# Autodesk Inventor assembly: 6_right_Arm_joint
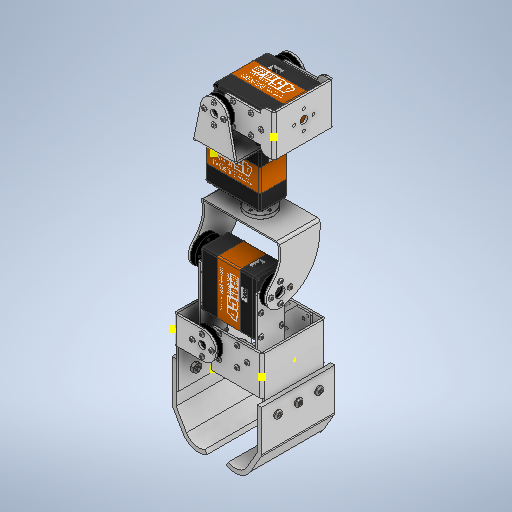
[picture p0: Inventor's stored thumbnail of the model, 512x512]
Saved by Autodesk Inventor 2026.1 (Build 301233020, 233B)
## iProperties
Created: 2026-01-04
Part Number: 6_right_Arm_joint
Document SubType Name: Assembly
Designer: aa992
Author: aa992
## Documents named in this file (18)
- C:\Users\aa992\OneDrive\Desktop\RHp_Humanoid_ver1\Assembly\6_right_Arm_joint.iam
- C:\Users\aa992\OneDrive\Desktop\RHp_Humanoid_ver1\Part\Frame\Arm\axis_18_top_frame.ipt
- C:\Users\aa992\OneDrive\Desktop\RHp_Humanoid_ver1\Part\HTD-45H, Horn\HTD-45H\HTD-45H.iam
- C:\Users\aa992\OneDrive\Desktop\RHp_Humanoid_ver1\Part\HTD-45H, Horn\Horn\Bottom Horn.ipt
- C:\Users\aa992\OneDrive\Desktop\RHp_Humanoid_ver1\Part\HTD-45H, Horn\Horn\Top Horn.ipt
- C:\Users\aa992\OneDrive\Desktop\RHp_Humanoid_ver1\Part\Frame\Arm\axis_19_bottom_frame.ipt
- C:\Users\aa992\OneDrive\Desktop\RHp_Humanoid_ver1\Part\HTD-45H, Horn\Horn\Top Horn silver.ipt
- C:\Users\aa992\OneDrive\Desktop\RHp_Humanoid_ver1\Part\Frame\Arm\axis_20_bottom_frame.ipt
- C:\Users\aa992\OneDrive\Desktop\RHp_Humanoid_ver1\Part\Frame\Arm\axis_21_top_frame.ipt
- C:\Users\aa992\OneDrive\Desktop\RHp_Humanoid_ver1\Part\Frame\Arm\axis_21_bottom_frame.ipt
- C:\Users\aa992\OneDrive\Desktop\RHp_Humanoid_ver1\Part\Frame\Arm\axis_22_top_frame.ipt
- C:\Users\aa992\OneDrive\Desktop\RHp_Humanoid_ver1\Part\Frame\Arm\axis_22_bottom_frame.ipt
- C:\Users\aa992\OneDrive\Desktop\RHp_Humanoid_ver1\Part\Frame\Arm\gripper_frame.ipt
- C:\Users\aa992\OneDrive\Desktop\RHp_Humanoid_ver1\Part\Bolt, Bearing, Nut, Washer\볼트, 너트\M2x4 Bolt.ipt
- C:\Users\aa992\OneDrive\Desktop\RHp_Humanoid_ver1\Part\Bolt, Bearing, Nut, Washer\볼트, 너트\M2x6 Bolt.ipt
- C:\Users\aa992\OneDrive\Desktop\RHp_Humanoid_ver1\Part\Bolt, Bearing, Nut, Washer\볼트, 너트\M3x6 Bolt.ipt
- C:\Users\aa992\OneDrive\Desktop\RHp_Humanoid_ver1\Part\Bolt, Bearing, Nut, Washer\볼트, 너트\M3 Nut.ipt
- C:\Users\aa992\OneDrive\Desktop\RHp_Humanoid_ver1\Part\Bolt, Bearing, Nut, Washer\볼트, 너트\M3x8 Bolt.ipt
## Components (99 placed, 17 different names)
1. axis_18_top_frame:1 — Flush:2, Mate:2, Flush:3, Rigid:1, Rigid:21, Rigid:22, Rigid:23, Rigid:24, Rigid:25, Rigid:26, Rigid:27, Rigid:28, Rigid:29
2. HTD-45H:1 [sub-assembly] — Rigid:1, Rotational:1, Rigid:2
3. Bottom Horn:1 — Rigid:2
4. Top Horn:1 — Rotational:1, Rigid:16
5. axis_19_bottom_frame:1 — Rigid:4, Rigid:16, Rigid:17, Rigid:18, Rigid:19, Rigid:20, Rigid:30, Rigid:31, Rigid:32, Rigid:33, Rigid:34, Rigid:35, Rigid:36, Rigid:37
6. HTD-45H:2 [sub-assembly] — Rigid:4, Rotational:2
7. Top Horn silver:1 — Rotational:2, Rigid:5
8. axis_20_bottom_frame:1 — Rigid:5, Rigid:6, Rigid:7, Rigid:38, Rigid:39, Rigid:40, Rigid:41, Rigid:42, Rigid:43, Rigid:44, Rigid:45, Rigid:46, Rigid:47, Rigid:48, Rigid:49
9. Top Horn:2 — Rigid:6, Rotational:3
10. Bottom Horn:2 — Rigid:7
11. HTD-45H:3 [sub-assembly] — Rotational:3, Rigid:8
12. axis_21_top_frame:1 — Rigid:8, Rigid:9, Rigid:50, Rigid:51, Rigid:52, Rigid:53, Rigid:54, Rigid:55, Rigid:56, Rigid:57, Rigid:58, Rigid:76, Rigid:77, Rigid:78, Rigid:79
13. axis_21_bottom_frame:1 — Rigid:9, Rigid:10, Rigid:12, Rigid:80, Rigid:81, Rigid:82, Rigid:83
14. HTD-45H:4 [sub-assembly] — Rigid:10, Rotational:4, Rigid:11
15. Top Horn:3 — Rotational:4, Rigid:13
16. Bottom Horn:3 — Rigid:11
17. axis_22_top_frame:1 — Rigid:12, Rigid:15, Rigid:63, Rigid:64, Rigid:65, Rigid:66, Rigid:67, Rigid:72, Rigid:73, Rigid:74, Rigid:75, Rigid:93, Rigid:94, Rigid:95
18. axis_22_bottom_frame:1 — Rigid:13, Rigid:14, Rigid:59, Rigid:60, Rigid:61, Rigid:62, Rigid:68, Rigid:69, Rigid:70, Rigid:71, Rigid:90, Rigid:91, Rigid:92
19. gripper_frame:1 — Rigid:14, Rigid:84, Rigid:85, Rigid:86
20. gripper_frame:2 — Rigid:15, Rigid:87, Rigid:88, Rigid:89
21. M2x4 Bolt:1 — Rigid:18
22. M2x4 Bolt:2 — Rigid:17
23. M2x4 Bolt:3 — Rigid:25
24. M2x4 Bolt:4 — Rigid:22
25. M2x4 Bolt:5 — Rigid:20
26. M2x4 Bolt:6 — Rigid:19
27. M2x4 Bolt:7 — Rigid:23
28. M2x4 Bolt:8 — Rigid:21
29. M2x4 Bolt:9 — Rigid:24
30. M2x4 Bolt:10 — Rigid:29
31. M2x4 Bolt:11 — Rigid:26
32. M2x4 Bolt:12 — Rigid:31
33. M2x4 Bolt:13 — Rigid:27
34. M2x4 Bolt:14 — Rigid:32
35. M2x4 Bolt:15 — Rigid:28
36. M2x4 Bolt:16 — Rigid:33
37. M2x4 Bolt:17 — Rigid:30
38. M2x4 Bolt:18 — Rigid:35
39. M2x4 Bolt:19 — Rigid:34
40. M2x4 Bolt:20 — Rigid:37
41. M2x4 Bolt:21 — Rigid:36
42. M2x4 Bolt:22 — Rigid:41
43. M2x4 Bolt:23 — Rigid:44
44. M2x4 Bolt:24 — Rigid:42
45. M2x4 Bolt:25 — Rigid:45
46. M2x4 Bolt:26 — Rigid:40
47. M2x4 Bolt:27 — Rigid:43
48. M2x4 Bolt:28 — Rigid:38
49. M2x4 Bolt:29 — Rigid:39
50. M2x4 Bolt:30 — Rigid:48
51. M2x4 Bolt:31 — Rigid:46
52. M2x4 Bolt:32 — Rigid:49
53. M2x4 Bolt:33 — Rigid:50
54. M2x4 Bolt:34 — Rigid:52
55. M2x4 Bolt:35 — Rigid:47
56. M2x4 Bolt:36 — Rigid:53
57. M2x4 Bolt:37 — Rigid:51
58. M2x4 Bolt:38 — Rigid:54
59. M2x4 Bolt:39 — Rigid:57
60. M2x4 Bolt:40 — Rigid:55
61. M2x4 Bolt:41 — Rigid:58
62. M2x4 Bolt:42 — Rigid:56
63. M2x4 Bolt:43 — Rigid:60
64. M2x4 Bolt:44 — Rigid:59
65. M2x4 Bolt:45 — Rigid:62
66. M2x4 Bolt:46 — Rigid:61
67. M2x6 Bolt:1 — Rigid:64
68. M2x6 Bolt:2 — Rigid:63
69. M2x6 Bolt:3 — Rigid:67
70. M2x6 Bolt:4 — Rigid:65
71. M2x6 Bolt:5 — Rigid:66
72. M2x4 Bolt:47 — Rigid:69
73. M2x4 Bolt:48 — Rigid:70
74. M2x4 Bolt:49 — Rigid:68
75. M2x4 Bolt:50 — Rigid:71
76. M2x6 Bolt:6 — Rigid:73
77. M2x6 Bolt:7 — Rigid:74
78. M2x6 Bolt:8 — Rigid:75
79. M2x6 Bolt:9 — Rigid:72
80. M3x6 Bolt:1 — Rigid:76
81. M3x6 Bolt:2 — Rigid:78
82. M3x6 Bolt:3 — Rigid:77
83. M3x6 Bolt:4 — Rigid:79
84. M3 Nut:1 — Rigid:80
85. M3 Nut:2 — Rigid:81
86. M3 Nut:3 — Rigid:82
87. M3 Nut:4 — Rigid:83
88. M3x8 Bolt:1 — Rigid:84
89. M3x8 Bolt:2 — Rigid:86
90. M3x8 Bolt:3 — Rigid:85
91. M3x8 Bolt:4 — Rigid:87
92. M3x8 Bolt:5 — Rigid:89
93. M3x8 Bolt:6 — Rigid:88
94. M3 Nut:5 — Rigid:91
95. M3 Nut:6 — Rigid:92
96. M3 Nut:7 — Rigid:90
97. M3 Nut:8 — Rigid:93
98. M3 Nut:9 — Rigid:94
99. M3 Nut:10 — Rigid:95
## Relationships (101: WeldJoint 94, RevoluteJoint 4, Flush 2, Mate 1)
- Flush:2: axis_18_top_frame:1
- Mate:2: axis_18_top_frame:1
- Flush:3: axis_18_top_frame:1
- Rigid:1 [WeldJoint]: axis_18_top_frame:1 ↔ HTD-45H:1
- Rotational:1 [RevoluteJoint]: HTD-45H:1 ↔ Top Horn:1
- Rigid:2 [WeldJoint]: HTD-45H:1 ↔ Bottom Horn:1
- Rigid:4 [WeldJoint]: axis_19_bottom_frame:1 ↔ HTD-45H:2
- Rotational:2 [RevoluteJoint]: HTD-45H:2 ↔ Top Horn silver:1
- Rigid:5 [WeldJoint]: Top Horn silver:1 ↔ axis_20_bottom_frame:1
- Rigid:6 [WeldJoint]: axis_20_bottom_frame:1 ↔ Top Horn:2
- Rigid:7 [WeldJoint]: axis_20_bottom_frame:1 ↔ Bottom Horn:2
- Rotational:3 [RevoluteJoint]: Top Horn:2 ↔ HTD-45H:3
- Rigid:8 [WeldJoint]: HTD-45H:3 ↔ axis_21_top_frame:1
- Rigid:9 [WeldJoint]: axis_21_top_frame:1 ↔ axis_21_bottom_frame:1
- Rigid:10 [WeldJoint]: axis_21_bottom_frame:1 ↔ HTD-45H:4
- Rotational:4 [RevoluteJoint]: HTD-45H:4 ↔ Top Horn:3
- Rigid:11 [WeldJoint]: HTD-45H:4 ↔ Bottom Horn:3
- Rigid:12 [WeldJoint]: axis_21_bottom_frame:1 ↔ axis_22_top_frame:1
- Rigid:13 [WeldJoint]: Top Horn:3 ↔ axis_22_bottom_frame:1
- Rigid:14 [WeldJoint]: axis_22_bottom_frame:1 ↔ gripper_frame:1
- Rigid:15 [WeldJoint]: axis_22_top_frame:1 ↔ gripper_frame:2
- Rigid:16 [WeldJoint]: Top Horn:1 ↔ axis_19_bottom_frame:1
- Rigid:17 [WeldJoint]: axis_19_bottom_frame:1 ↔ M2x4 Bolt:2
- Rigid:18 [WeldJoint]: axis_19_bottom_frame:1 ↔ M2x4 Bolt:1
- Rigid:19 [WeldJoint]: axis_19_bottom_frame:1 ↔ M2x4 Bolt:6
- Rigid:20 [WeldJoint]: axis_19_bottom_frame:1 ↔ M2x4 Bolt:5
- Rigid:21 [WeldJoint]: axis_18_top_frame:1 ↔ M2x4 Bolt:8
- Rigid:22 [WeldJoint]: axis_18_top_frame:1 ↔ M2x4 Bolt:4
- Rigid:23 [WeldJoint]: axis_18_top_frame:1 ↔ M2x4 Bolt:7
- Rigid:24 [WeldJoint]: axis_18_top_frame:1 ↔ M2x4 Bolt:9
- Rigid:25 [WeldJoint]: axis_18_top_frame:1 ↔ M2x4 Bolt:3
- Rigid:26 [WeldJoint]: axis_18_top_frame:1 ↔ M2x4 Bolt:11
- Rigid:27 [WeldJoint]: axis_18_top_frame:1 ↔ M2x4 Bolt:13
- Rigid:28 [WeldJoint]: axis_18_top_frame:1 ↔ M2x4 Bolt:15
- Rigid:29 [WeldJoint]: axis_18_top_frame:1 ↔ M2x4 Bolt:10
- Rigid:30 [WeldJoint]: axis_19_bottom_frame:1 ↔ M2x4 Bolt:17
- Rigid:31 [WeldJoint]: axis_19_bottom_frame:1 ↔ M2x4 Bolt:12
- Rigid:32 [WeldJoint]: axis_19_bottom_frame:1 ↔ M2x4 Bolt:14
- Rigid:33 [WeldJoint]: axis_19_bottom_frame:1 ↔ M2x4 Bolt:16
- Rigid:34 [WeldJoint]: axis_19_bottom_frame:1 ↔ M2x4 Bolt:19
- Rigid:35 [WeldJoint]: axis_19_bottom_frame:1 ↔ M2x4 Bolt:18
- Rigid:36 [WeldJoint]: axis_19_bottom_frame:1 ↔ M2x4 Bolt:21
- Rigid:37 [WeldJoint]: axis_19_bottom_frame:1 ↔ M2x4 Bolt:20
- Rigid:38 [WeldJoint]: axis_20_bottom_frame:1 ↔ M2x4 Bolt:28
- Rigid:39 [WeldJoint]: axis_20_bottom_frame:1 ↔ M2x4 Bolt:29
- Rigid:40 [WeldJoint]: axis_20_bottom_frame:1 ↔ M2x4 Bolt:26
- Rigid:41 [WeldJoint]: axis_20_bottom_frame:1 ↔ M2x4 Bolt:22
- Rigid:42 [WeldJoint]: axis_20_bottom_frame:1 ↔ M2x4 Bolt:24
- Rigid:43 [WeldJoint]: axis_20_bottom_frame:1 ↔ M2x4 Bolt:27
- Rigid:44 [WeldJoint]: axis_20_bottom_frame:1 ↔ M2x4 Bolt:23
- Rigid:45 [WeldJoint]: axis_20_bottom_frame:1 ↔ M2x4 Bolt:25
- Rigid:46 [WeldJoint]: axis_20_bottom_frame:1 ↔ M2x4 Bolt:31
- Rigid:47 [WeldJoint]: axis_20_bottom_frame:1 ↔ M2x4 Bolt:35
- Rigid:48 [WeldJoint]: axis_20_bottom_frame:1 ↔ M2x4 Bolt:30
- Rigid:49 [WeldJoint]: axis_20_bottom_frame:1 ↔ M2x4 Bolt:32
- Rigid:50 [WeldJoint]: axis_21_top_frame:1 ↔ M2x4 Bolt:33
- Rigid:51 [WeldJoint]: axis_21_top_frame:1 ↔ M2x4 Bolt:37
- Rigid:52 [WeldJoint]: axis_21_top_frame:1 ↔ M2x4 Bolt:34
- Rigid:53 [WeldJoint]: axis_21_top_frame:1 ↔ M2x4 Bolt:36
- Rigid:54 [WeldJoint]: axis_21_top_frame:1 ↔ M2x4 Bolt:38
- Rigid:55 [WeldJoint]: axis_21_top_frame:1 ↔ M2x4 Bolt:40
- Rigid:56 [WeldJoint]: axis_21_top_frame:1 ↔ M2x4 Bolt:42
- Rigid:57 [WeldJoint]: axis_21_top_frame:1 ↔ M2x4 Bolt:39
- Rigid:58 [WeldJoint]: axis_21_top_frame:1 ↔ M2x4 Bolt:41
- Rigid:59 [WeldJoint]: axis_22_bottom_frame:1 ↔ M2x4 Bolt:44
- Rigid:60 [WeldJoint]: axis_22_bottom_frame:1 ↔ M2x4 Bolt:43
- Rigid:61 [WeldJoint]: axis_22_bottom_frame:1 ↔ M2x4 Bolt:46
- Rigid:62 [WeldJoint]: axis_22_bottom_frame:1 ↔ M2x4 Bolt:45
- Rigid:63 [WeldJoint]: axis_22_top_frame:1 ↔ M2x6 Bolt:2
- Rigid:64 [WeldJoint]: axis_22_top_frame:1 ↔ M2x6 Bolt:1
- Rigid:65 [WeldJoint]: axis_22_top_frame:1 ↔ M2x6 Bolt:4
- Rigid:66 [WeldJoint]: axis_22_top_frame:1 ↔ M2x6 Bolt:5
- Rigid:67 [WeldJoint]: axis_22_top_frame:1 ↔ M2x6 Bolt:3
- Rigid:68 [WeldJoint]: axis_22_bottom_frame:1 ↔ M2x4 Bolt:49
- Rigid:69 [WeldJoint]: axis_22_bottom_frame:1 ↔ M2x4 Bolt:47
- Rigid:70 [WeldJoint]: axis_22_bottom_frame:1 ↔ M2x4 Bolt:48
- Rigid:71 [WeldJoint]: axis_22_bottom_frame:1 ↔ M2x4 Bolt:50
- Rigid:72 [WeldJoint]: axis_22_top_frame:1 ↔ M2x6 Bolt:9
- Rigid:73 [WeldJoint]: axis_22_top_frame:1 ↔ M2x6 Bolt:6
- Rigid:74 [WeldJoint]: axis_22_top_frame:1 ↔ M2x6 Bolt:7
- Rigid:75 [WeldJoint]: axis_22_top_frame:1 ↔ M2x6 Bolt:8
- Rigid:76 [WeldJoint]: axis_21_top_frame:1 ↔ M3x6 Bolt:1
- Rigid:77 [WeldJoint]: axis_21_top_frame:1 ↔ M3x6 Bolt:3
- Rigid:78 [WeldJoint]: axis_21_top_frame:1 ↔ M3x6 Bolt:2
- Rigid:79 [WeldJoint]: axis_21_top_frame:1 ↔ M3x6 Bolt:4
- Rigid:80 [WeldJoint]: axis_21_bottom_frame:1 ↔ M3 Nut:1
- Rigid:81 [WeldJoint]: axis_21_bottom_frame:1 ↔ M3 Nut:2
- Rigid:82 [WeldJoint]: axis_21_bottom_frame:1 ↔ M3 Nut:3
- Rigid:83 [WeldJoint]: axis_21_bottom_frame:1 ↔ M3 Nut:4
- Rigid:84 [WeldJoint]: gripper_frame:1 ↔ M3x8 Bolt:1
- Rigid:85 [WeldJoint]: gripper_frame:1 ↔ M3x8 Bolt:3
- Rigid:86 [WeldJoint]: gripper_frame:1 ↔ M3x8 Bolt:2
- Rigid:87 [WeldJoint]: gripper_frame:2 ↔ M3x8 Bolt:4
- Rigid:88 [WeldJoint]: gripper_frame:2 ↔ M3x8 Bolt:6
- Rigid:89 [WeldJoint]: gripper_frame:2 ↔ M3x8 Bolt:5
- Rigid:90 [WeldJoint]: axis_22_bottom_frame:1 ↔ M3 Nut:7
- Rigid:91 [WeldJoint]: axis_22_bottom_frame:1 ↔ M3 Nut:5
- Rigid:92 [WeldJoint]: axis_22_bottom_frame:1 ↔ M3 Nut:6
- Rigid:93 [WeldJoint]: axis_22_top_frame:1 ↔ M3 Nut:8
- Rigid:94 [WeldJoint]: axis_22_top_frame:1 ↔ M3 Nut:9
- Rigid:95 [WeldJoint]: axis_22_top_frame:1 ↔ M3 Nut:10
